# Autodesk Inventor assembly: Assembly2
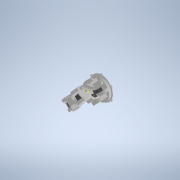
[picture p0: Inventor's stored thumbnail of the model, 180x180]
Saved by Autodesk Inventor 2022 (Build 260153000, 153)
## iProperties
Created: 2022-01-07
Part Number: Assembly2
Document SubType Name: Assembly
Designer: nguye
Author: nguye
## Documents named in this file (9)
- G:\My Drive\Study\Semester 5\Roboty Uslugowe\Project\Model\Assembly2.iam
- G:\My Drive\Study\Semester 5\Roboty Uslugowe\Project\Model\Base.ipt
- G:\My Drive\Study\Semester 5\Roboty Uslugowe\Project\Model\Baserotate.ipt
- G:\My Drive\Study\Semester 5\Roboty Uslugowe\Project\Model\Servo.ipt
- G:\My Drive\Study\Semester 5\Roboty Uslugowe\Project\Model\Foot.ipt
- G:\My Drive\Study\Semester 5\Roboty Uslugowe\Project\Model\PartArmNEW.ipt
- G:\My Drive\Study\Semester 5\Roboty Uslugowe\Project\Model\PartArm1.ipt
- G:\My Drive\Study\Semester 5\Roboty Uslugowe\Project\Model\Grippera.iam
- G:\My Drive\Study\Semester 5\Roboty Uslugowe\Project\Model\Servosmall.ipt
## Components (15 placed, 8 different names)
1. Base:1 — Mate:4, Mate:5
2. Baserotate:1 — Mate:1, Mate:2, Mate:3, Mate:6, Mate:7, Mate:8, Mate:9, Mate:10, Mate:11
3. Servo:1 — Mate:1, Mate:2, Mate:3, Mate:4, Mate:5
4. Foot:1 — Mate:6, Mate:7, Mate:8, Mate:13, Mate:34
5. Foot:2 — Mate:9, Mate:10, Mate:11, Mate:12
6. PartArmNEW:1 — Mate:12, Mate:13, Mate:14, Mate:15, Mate:22, Mate:23, Mate:24
7. PartArmNEW:2 — Mate:14, Mate:15, Mate:16, Mate:17, Mate:25, Mate:26, Mate:27
8. PartArmNEW:3 — Mate:16, Mate:17, Mate:18, Mate:19, Mate:28, Mate:29, Mate:30
9. PartArm1:1 — Mate:18, Mate:19, Mate:20, Mate:21, Mate:31, Mate:32, Mate:33
10. Grippera:1 [sub-assembly] — Mate:20, Mate:21
11. Servosmall:1 — Mate:22, Mate:23, Mate:24
12. Servosmall:2 — Mate:25, Mate:26, Mate:27
13. Servosmall:3 — Mate:28, Mate:29, Mate:30
14. Servosmall:4 — Mate:31, Mate:32, Mate:33
15. Servosmall:5 — Mate:34
## Relationships (34: Mate 34)
- Mate:1: Baserotate:1 ↔ Servo:1
- Mate:2: Baserotate:1 ↔ Servo:1
- Mate:3: Baserotate:1 ↔ Servo:1
- Mate:4: Base:1 ↔ Servo:1
- Mate:5: Base:1 ↔ Servo:1
- Mate:6: Baserotate:1 ↔ Foot:1
- Mate:7: Baserotate:1 ↔ Foot:1
- Mate:8: Baserotate:1 ↔ Foot:1
- Mate:9: Baserotate:1 ↔ Foot:2
- Mate:10: Baserotate:1 ↔ Foot:2
- Mate:11: Baserotate:1 ↔ Foot:2
- Mate:12: Foot:2 ↔ PartArmNEW:1
- Mate:13: Foot:1 ↔ PartArmNEW:1
- Mate:14: PartArmNEW:1 ↔ PartArmNEW:2
- Mate:15: PartArmNEW:1 ↔ PartArmNEW:2
- Mate:16: PartArmNEW:2 ↔ PartArmNEW:3
- Mate:17: PartArmNEW:2 ↔ PartArmNEW:3
- Mate:18: PartArmNEW:3 ↔ PartArm1:1
- Mate:19: PartArmNEW:3 ↔ PartArm1:1
- Mate:20: PartArm1:1 ↔ Grippera:1
- Mate:21: PartArm1:1 ↔ Grippera:1
- Mate:22: PartArmNEW:1 ↔ Servosmall:1
- Mate:23: PartArmNEW:1 ↔ Servosmall:1
- Mate:24: PartArmNEW:1 ↔ Servosmall:1
- Mate:25: PartArmNEW:2 ↔ Servosmall:2
- Mate:26: PartArmNEW:2 ↔ Servosmall:2
- Mate:27: PartArmNEW:2 ↔ Servosmall:2
- Mate:28: PartArmNEW:3 ↔ Servosmall:3
- Mate:29: PartArmNEW:3 ↔ Servosmall:3
- Mate:30: PartArmNEW:3 ↔ Servosmall:3
- Mate:31: PartArm1:1 ↔ Servosmall:4
- Mate:32: PartArm1:1 ↔ Servosmall:4
- Mate:33: PartArm1:1 ↔ Servosmall:4
- Mate:34: Foot:1 ↔ Servosmall:5
